# Autodesk Inventor assembly: G assembly
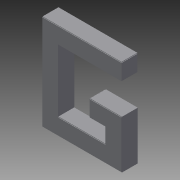
[picture p0: Inventor's stored thumbnail of the model, 180x180]
Saved by Autodesk Inventor 2013 (Build 170138000, 138)
## iProperties
Created: 2014-03-22
Part Number: G assembly
Document SubType Name: Assembly
Designer: kahohbein
Author: kahohbein
## Documents named in this file (10)
- C:\Users\kahohbein\Documents\GitHub\2013-2014_BlockParty\CAD\Hangar Project\G assembly.iam
- C:\Users\kahohbein\Documents\GitHub\2013-2014_BlockParty\CAD\Hangar Project\G face.ipt
- C:\Users\kahohbein\Documents\GitHub\2013-2014_BlockParty\CAD\Hangar Project\G  small side x4.ipt
- C:\Users\kahohbein\Documents\GitHub\2013-2014_BlockParty\CAD\Hangar Project\G inside bottom.ipt
- C:\Users\kahohbein\Documents\GitHub\2013-2014_BlockParty\CAD\Hangar Project\G inside lip top.ipt
- C:\Users\kahohbein\Documents\GitHub\2013-2014_BlockParty\CAD\Hangar Project\G inside side.ipt
- C:\Users\kahohbein\Documents\GitHub\2013-2014_BlockParty\CAD\Hangar Project\G inside top.ipt
- C:\Users\kahohbein\Documents\GitHub\2013-2014_BlockParty\CAD\Hangar Project\G long side.ipt
- C:\Users\kahohbein\Documents\GitHub\2013-2014_BlockParty\CAD\Hangar Project\G side.ipt
- C:\Users\kahohbein\Documents\GitHub\2013-2014_BlockParty\CAD\Hangar Project\G topbottom x2.ipt
## Components (13 placed, 9 different names)
1. G face:1 — Mate:1, Mate:2, Mate:3, Mate:6, Mate:8, Mate:10, Mate:12, Mate:14, Mate:17, Mate:19, Mate:20, Mate:25
2. G  small side x4:1 — Mate:2, Mate:5, Mate:11
3. G  small side x4:2 — Mate:3, Mate:5, Mate:7
4. G  small side x4:3 — Mate:1, Mate:16, Mate:21
5. G  small side x4:4 — Mate:6, Mate:7, Mate:9
6. G inside bottom:1 — Mate:8, Mate:9, Mate:13
7. G inside lip top:1 — Mate:10, Mate:11, Mate:24
8. G inside side:1 — Mate:12, Mate:13, Mate:15, Flush:1
9. G inside top:1 — Mate:14, Mate:15, Flush:1, Mate:16
10. G long side:1 — Mate:17, Mate:22, Mate:23
11. G side:1 — Mate:24, Mate:25
12. G topbottom x2:1 — Mate:19, Mate:21, Mate:22
13. G topbottom x2:2 — Mate:20, Mate:23
## Relationships (24: Mate 23, Flush 1)
- Mate:1: G face:1 ↔ G  small side x4:3
- Mate:2: G face:1 ↔ G  small side x4:1
- Mate:3: G face:1 ↔ G  small side x4:2
- Mate:5: G  small side x4:1 ↔ G  small side x4:2
- Mate:6: G face:1 ↔ G  small side x4:4
- Mate:7: G  small side x4:2 ↔ G  small side x4:4
- Mate:8: G face:1 ↔ G inside bottom:1
- Mate:9: G  small side x4:4 ↔ G inside bottom:1
- Mate:10: G face:1 ↔ G inside lip top:1
- Mate:11: G  small side x4:1 ↔ G inside lip top:1
- Mate:12: G face:1 ↔ G inside side:1
- Mate:13: G inside bottom:1 ↔ G inside side:1
- Mate:14: G face:1 ↔ G inside top:1
- Mate:15: G inside side:1 ↔ G inside top:1
- Flush:1: G inside side:1 ↔ G inside top:1
- Mate:16: G  small side x4:3 ↔ G inside top:1
- Mate:17: G face:1 ↔ G long side:1
- Mate:19: G face:1 ↔ G topbottom x2:1
- Mate:20: G face:1 ↔ G topbottom x2:2
- Mate:21: G  small side x4:3 ↔ G topbottom x2:1
- Mate:22: G long side:1 ↔ G topbottom x2:1
- Mate:23: G long side:1 ↔ G topbottom x2:2
- Mate:24: G inside lip top:1 ↔ G side:1
- Mate:25: G face:1 ↔ G side:1
